# Autodesk Inventor assembly: Assy_foot
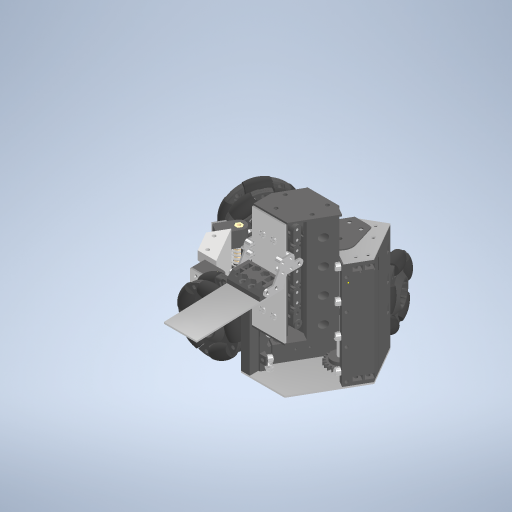
[picture p0: Inventor's stored thumbnail of the model, 512x512]
Saved by Autodesk Inventor 2024.1 (Build 281209000, 209)
## iProperties
Created: 2025-02-03
Part Number: Assy_foot
Document SubType Name: Assembly
Designer: hibik
Author: hibik
## Documents named in this file (4)
- C:\Users\hibik\Documents\Robomech\RESCUE\ORCA\hard\Assy_foot.iam
- C:\Users\hibik\Documents\Robomech\RESCUE\ORCA\hard\flame_base\base.iam
- C:\Users\hibik\Documents\Robomech\RESCUE\ORCA\hard\omni_wheel\Assy_omni_wheel.iam
- C:\Users\hibik\Documents\Robomech\RESCUE\ORCA\hard\fork\right\Assy_fork_right.iam
## Components (5 placed, 3 different names)
1. base:1 [sub-assembly] — 挿入:1, 挿入:2, 挿入:3, 挿入:4, 挿入:5, 挿入:6
2. Assy_omni_wheel:1 [sub-assembly] — 挿入:1, 挿入:2
3. Assy_omni_wheel:2 [sub-assembly] — 挿入:3, 挿入:4
4. Assy_omni_wheel:3 [sub-assembly] — 挿入:5, 挿入:6
5. Assy_fork_right:1 [sub-assembly]
## Relationships (6: Insert 6)
- 挿入:1 [Insert]: base:1 ↔ Assy_omni_wheel:1
- 挿入:2 [Insert]: base:1 ↔ Assy_omni_wheel:1
- 挿入:3 [Insert]: base:1 ↔ Assy_omni_wheel:2
- 挿入:4 [Insert]: base:1 ↔ Assy_omni_wheel:2
- 挿入:5 [Insert]: base:1 ↔ Assy_omni_wheel:3
- 挿入:6 [Insert]: base:1 ↔ Assy_omni_wheel:3
